# Autodesk Inventor assembly: Passion-v2
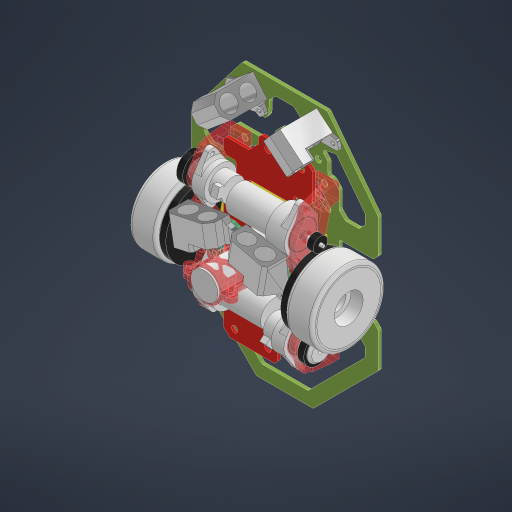
[picture p0: Inventor's stored thumbnail of the model, 512x512]
Saved by Autodesk Inventor 2023.5 (Build 275446000, 446)
## iProperties
Created: 2025-01-19
Part Number: Passion-v2
Document SubType Name: Assembly
Designer: IshiiLabHonda
Author: IshiiLabHonda
## Documents named in this file (23)
- C:\Users\IshiiLabHonda\Documents\Micromouse\Passion-v2\Inventor\Passion-v2-3\Passion-v2.iam
- C:\Users\IshiiLabHonda\Documents\Micromouse\Passion-v2\Inventor\Passion-v2-3\Origin\chassis.ipt
- C:\Users\IshiiLabHonda\Documents\Micromouse\Passion-v2\Inventor\Passion-v2-3\Readymade\Motor-8520.ipt
- C:\Users\IshiiLabHonda\Documents\Micromouse\Passion-v2\Inventor\Passion-v2-3\Readymade\Encoder-7S-400-2MC-50-00E.ipt
- C:\Users\IshiiLabHonda\Documents\Micromouse\Passion-v2\Inventor\Passion-v2-3\Readymade\Pinion-Gear_M0.3_15T.ipt
- C:\Users\IshiiLabHonda\Documents\Micromouse\Passion-v2\Inventor\Passion-v2-3\Readymade\Encoder-Gear_M0.3_29T.ipt
- C:\Users\IshiiLabHonda\Documents\Micromouse\Passion-v2\Inventor\Passion-v2-3\Readymade\Spur-Gear_M0.3_71T_t2.0_D8.ipt
- C:\Users\IshiiLabHonda\Documents\Micromouse\Passion-v2\Inventor\Passion-v2-3\Readymade\Wheel_MZH131W-N2.ipt
- C:\Users\IshiiLabHonda\Documents\Micromouse\Passion-v2\Inventor\Passion-v2-3\Readymade\Tire-MZW39-40.ipt
- C:\Users\IshiiLabHonda\Documents\Micromouse\Passion-v2\Inventor\Passion-v2-3\Readymade\Encoder-Gear-Spacer.ipt
- C:\Users\IshiiLabHonda\Documents\Micromouse\Passion-v2\Inventor\Passion-v2-3\Origin\motormount-r.ipt
- C:\Users\IshiiLabHonda\Documents\Micromouse\Passion-v2\Inventor\Passion-v2-3\Origin\motormount-l.ipt
- C:\Users\IshiiLabHonda\Documents\Micromouse\Passion-v2\Inventor\Passion-v2-3\Common\spacer-outwheel-m3-1.ipt
- C:\Users\IshiiLabHonda\Documents\Micromouse\Passion-v2\Inventor\Passion-v2-3\Origin\circuit.ipt
- C:\Users\IshiiLabHonda\Documents\Micromouse\Passion-v2\Inventor\Passion-v2-3\Origin\encodersupporter.ipt
- C:\Users\IshiiLabHonda\Documents\Micromouse\Passion-v2\Inventor\Passion-v2-3\Origin\sensormount.ipt
- C:\Users\IshiiLabHonda\Documents\Micromouse\Passion-v2\Inventor\Passion-v2-3\Origin\motorsupporter.ipt
- C:\Users\IshiiLabHonda\Documents\Micromouse\Passion-v2\Inventor\Passion-v2-3\Origin\sensorbase.ipt
- C:\Users\IshiiLabHonda\Documents\Micromouse\Passion-v2\Inventor\Passion-v2-3\Origin\frontsensorholder.ipt
- C:\Users\IshiiLabHonda\Documents\Micromouse\Passion-v2\Inventor\Passion-v2-3\Origin\fanmotor-mount-1.ipt
- C:\Users\IshiiLabHonda\Documents\Micromouse\Passion-v2\Inventor\Passion-v2-3\Origin\fanmotor-mount-2.ipt
- C:\Users\IshiiLabHonda\Documents\Micromouse\Passion-v2\Inventor\Passion-v2-3\Origin\fanmotor-mount-2-1.ipt
- C:\Users\IshiiLabHonda\Documents\Micromouse\Passion-v2\Inventor\Passion-v2-3\Origin\fan-concreate.ipt
## Components (34 placed, 22 different names)
1. chassis:1 — フラッシュ:1, メイト:1, メイト:2, メイト:37, メイト:43, メイト:71, メイト:82, メイト:103, メイト:111, メイト:112, メイト:115, メイト:121, メイト:122, メイト:135
2. Motor-8520:1 — メイト:12, メイト:44, メイト:87, メイト:104
3. Encoder-7S-400-2MC-50-00E:1 — メイト:13, メイト:50, メイト:61, メイト:110
4. Pinion-Gear_M0.3_15T:1 — メイト:12, フラッシュ:7
5. Encoder-Gear_M0.3_29T:1 — メイト:13, メイト:18, メイト:19, フラッシュ:6
6. Spur-Gear_M0.3_71T_t2.0_D8:1 — メイト:17, メイト:59, フラッシュ:6, フラッシュ:7
7. Wheel_MZH131W-N2:1 — メイト:15, フラッシュ:2, メイト:17, メイト:56, メイト:59, メイト:60
8. Tire-MZW39-40:1 — メイト:15, フラッシュ:2
9. Encoder-Gear-Spacer:1 — メイト:18, メイト:19
10. motormount-r:1 — メイト:37, メイト:38, メイト:39, メイト:40, メイト:111, メイト:112, メイト:113, メイト:116, メイト:117, メイト:118, メイト:119, メイト:120, メイト:128
11. Encoder-7S-400-2MC-50-00E:2 — メイト:34, メイト:39, メイト:65, メイト:128
12. Motor-8520:2 — メイト:33, メイト:40, メイト:88
13. Spur-Gear_M0.3_71T_t2.0_D8:2 — メイト:29, フラッシュ:4, フラッシュ:5
14. Wheel_MZH131W-N2:2 — メイト:29, メイト:38, メイト:48
15. Tire-MZW39-40:2 — メイト:46
16. Pinion-Gear_M0.3_15T:2 — メイト:33, フラッシュ:4
17. Encoder-Gear_M0.3_29T:2 — メイト:34, フラッシュ:5
18. Encoder-Gear-Spacer:2
19. motormount-l:1 — メイト:43, メイト:44, メイト:50, メイト:58, メイト:89, メイト:91, メイト:94, メイト:98, メイト:99, メイト:102, メイト:103, メイト:104, メイト:105, メイト:110, メイト:114
20. spacer-outwheel-m3-1:1 — メイト:46, メイト:48
21. Motor-8520:3 — メイト:82, メイト:100, メイト:101, メイト:125, メイト:130, メイト:132, メイト:134
22. circuit:1 — メイト:100, メイト:101, メイト:102, メイト:115, メイト:126, メイト:127
23. spacer-outwheel-m3-1:2 — メイト:56, メイト:58, メイト:60, メイト:98, メイト:99
24. encodersupporter:1 — メイト:61, メイト:91, メイト:105
25. encodersupporter:4 — メイト:65, メイト:119, メイト:120
26. sensormount:1 — メイト:71, メイト:121, メイト:122
27. motorsupporter:1 — メイト:87, メイト:89
28. motorsupporter:2 — メイト:88, メイト:116, メイト:117, メイト:118
29. sensorbase:1 — メイト:94, メイト:97, メイト:113, メイト:114, メイト:123, メイト:124, メイト:129, メイト:131
30. frontsensorholder:1 — メイト:97, メイト:123, メイト:124
31. fanmotor-mount-1:1 — メイト:125, メイト:126, メイト:127
32. fanmotor-mount-2:1 — メイト:129, メイト:130, メイト:131, メイト:133
33. fanmotor-mount-2-1:1 — メイト:132, メイト:133
34. fan-concreate:1 — メイト:134, メイト:135
## Relationships (79: Mate 72, Flush 7)
- フラッシュ:1 [Flush]: chassis:1
- メイト:1 [Mate]: chassis:1
- メイト:2 [Mate]: chassis:1
- メイト:12 [Mate]: Motor-8520:1 ↔ Pinion-Gear_M0.3_15T:1
- メイト:13 [Mate]: Encoder-7S-400-2MC-50-00E:1 ↔ Encoder-Gear_M0.3_29T:1
- メイト:15 [Mate]: Wheel_MZH131W-N2:1 ↔ Tire-MZW39-40:1
- フラッシュ:2 [Flush]: Wheel_MZH131W-N2:1 ↔ Tire-MZW39-40:1
- メイト:17 [Mate]: Spur-Gear_M0.3_71T_t2.0_D8:1 ↔ Wheel_MZH131W-N2:1
- メイト:18 [Mate]: Encoder-Gear_M0.3_29T:1 ↔ Encoder-Gear-Spacer:1
- メイト:19 [Mate]: Encoder-Gear_M0.3_29T:1 ↔ Encoder-Gear-Spacer:1
- [Mate]: Wheel_MZH131W-N2:2 ↔ Tire-MZW39-40:2
- [Flush]: Wheel_MZH131W-N2:2 ↔ Tire-MZW39-40:2
- [Mate]: Spur-Gear_M0.3_71T_t2.0_D8:2 ↔ Wheel_MZH131W-N2:2
- メイト:29 [Mate]: Spur-Gear_M0.3_71T_t2.0_D8:2 ↔ Wheel_MZH131W-N2:2
- [Mate]: Encoder-Gear_M0.3_29T:2 ↔ Encoder-Gear-Spacer:2
- [Mate]: Encoder-Gear_M0.3_29T:2 ↔ Encoder-Gear-Spacer:2
- メイト:33 [Mate]: Motor-8520:2 ↔ Pinion-Gear_M0.3_15T:2
- メイト:34 [Mate]: Encoder-7S-400-2MC-50-00E:2 ↔ Encoder-Gear_M0.3_29T:2
- メイト:37 [Mate]: chassis:1 ↔ motormount-r:1
- メイト:38 [Mate]: motormount-r:1 ↔ Wheel_MZH131W-N2:2
- メイト:39 [Mate]: motormount-r:1 ↔ Encoder-7S-400-2MC-50-00E:2
- メイト:40 [Mate]: motormount-r:1 ↔ Motor-8520:2
- メイト:43 [Mate]: chassis:1 ↔ motormount-l:1
- メイト:44 [Mate]: Motor-8520:1 ↔ motormount-l:1
- メイト:46 [Mate]: Tire-MZW39-40:2 ↔ spacer-outwheel-m3-1:1
- メイト:48 [Mate]: Wheel_MZH131W-N2:2 ↔ spacer-outwheel-m3-1:1
- フラッシュ:4 [Flush]: Spur-Gear_M0.3_71T_t2.0_D8:2 ↔ Pinion-Gear_M0.3_15T:2
- フラッシュ:5 [Flush]: Spur-Gear_M0.3_71T_t2.0_D8:2 ↔ Encoder-Gear_M0.3_29T:2
- メイト:50 [Mate]: Encoder-7S-400-2MC-50-00E:1 ↔ motormount-l:1
- メイト:56 [Mate]: Wheel_MZH131W-N2:1 ↔ spacer-outwheel-m3-1:2
- メイト:58 [Mate]: motormount-l:1 ↔ spacer-outwheel-m3-1:2
- メイト:59 [Mate]: Spur-Gear_M0.3_71T_t2.0_D8:1 ↔ Wheel_MZH131W-N2:1
- メイト:60 [Mate]: Wheel_MZH131W-N2:1 ↔ spacer-outwheel-m3-1:2
- メイト:61 [Mate]: Encoder-7S-400-2MC-50-00E:1 ↔ encodersupporter:1
- メイト:65 [Mate]: Encoder-7S-400-2MC-50-00E:2 ↔ encodersupporter:4
- メイト:71 [Mate]: chassis:1 ↔ sensormount:1
- メイト:82 [Mate]: chassis:1 ↔ Motor-8520:3
- フラッシュ:6 [Flush]: Encoder-Gear_M0.3_29T:1 ↔ Spur-Gear_M0.3_71T_t2.0_D8:1
- フラッシュ:7 [Flush]: Pinion-Gear_M0.3_15T:1 ↔ Spur-Gear_M0.3_71T_t2.0_D8:1
- メイト:87 [Mate]: Motor-8520:1 ↔ motorsupporter:1
- メイト:88 [Mate]: Motor-8520:2 ↔ motorsupporter:2
- メイト:89 [Mate]: motormount-l:1 ↔ motorsupporter:1
- メイト:91 [Mate]: motormount-l:1 ↔ encodersupporter:1
- メイト:94 [Mate]: motormount-l:1 ↔ sensorbase:1
- メイト:97 [Mate]: sensorbase:1 ↔ frontsensorholder:1
- メイト:98 [Mate]: motormount-l:1 ↔ spacer-outwheel-m3-1:2
- メイト:99 [Mate]: motormount-l:1 ↔ spacer-outwheel-m3-1:2
- メイト:100 [Mate]: Motor-8520:3 ↔ circuit:1
- メイト:101 [Mate]: Motor-8520:3 ↔ circuit:1
- メイト:102 [Mate] (0.5 mm): motormount-l:1 ↔ circuit:1
- メイト:103 [Mate]: chassis:1 ↔ motormount-l:1
- メイト:104 [Mate]: Motor-8520:1 ↔ motormount-l:1
- メイト:105 [Mate]: motormount-l:1 ↔ encodersupporter:1
- メイト:110 [Mate]: Encoder-7S-400-2MC-50-00E:1 ↔ motormount-l:1
- メイト:111 [Mate]: chassis:1 ↔ motormount-r:1
- メイト:112 [Mate]: chassis:1 ↔ motormount-r:1
- メイト:113 [Mate]: motormount-r:1 ↔ sensorbase:1
- メイト:114 [Mate]: motormount-l:1 ↔ sensorbase:1
- メイト:115 [Mate] (4.5 mm): chassis:1 ↔ circuit:1
- メイト:116 [Mate]: motormount-r:1 ↔ motorsupporter:2
- メイト:117 [Mate]: motormount-r:1 ↔ motorsupporter:2
- メイト:118 [Mate]: motormount-r:1 ↔ motorsupporter:2
- メイト:119 [Mate]: motormount-r:1 ↔ encodersupporter:4
- メイト:120 [Mate]: motormount-r:1 ↔ encodersupporter:4
- メイト:121 [Mate]: chassis:1 ↔ sensormount:1
- メイト:122 [Mate]: chassis:1 ↔ sensormount:1
- メイト:123 [Mate]: sensorbase:1 ↔ frontsensorholder:1
- メイト:124 [Mate]: sensorbase:1 ↔ frontsensorholder:1
- メイト:125 [Mate]: Motor-8520:3 ↔ fanmotor-mount-1:1
- メイト:126 [Mate]: circuit:1 ↔ fanmotor-mount-1:1
- メイト:127 [Mate]: circuit:1 ↔ fanmotor-mount-1:1
- メイト:128 [Mate]: motormount-r:1 ↔ Encoder-7S-400-2MC-50-00E:2
- メイト:129 [Mate]: sensorbase:1 ↔ fanmotor-mount-2:1
- メイト:130 [Mate]: Motor-8520:3 ↔ fanmotor-mount-2:1
- メイト:131 [Mate]: sensorbase:1 ↔ fanmotor-mount-2:1
- メイト:132 [Mate]: Motor-8520:3 ↔ fanmotor-mount-2-1:1
- メイト:133 [Mate]: fanmotor-mount-2:1 ↔ fanmotor-mount-2-1:1
- メイト:134 [Mate]: Motor-8520:3 ↔ fan-concreate:1
- メイト:135 [Mate] (0.5 mm): chassis:1 ↔ fan-concreate:1
## Named parameters: d41_d25 = 0 mm, d42_d26 = 0 mm, d43_d28 = 0 mm, d46_d29 = 0 mm, d47_d30 = 0 mm
